# Autodesk Inventor assembly: Assembly1
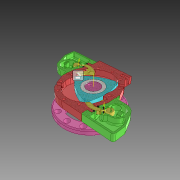
[picture p0: Inventor's stored thumbnail of the model, 180x180]
Saved by Autodesk Inventor 2020 (Build 240168000, 168)
## iProperties
Created: 2021-01-24
Part Number: Assembly1
Document SubType Name: Assembly
Designer: DDeGo
Author: DDeGo
## Documents named in this file (15)
- C:\Users\DDeGo\Documents\Drew\Projects\AirWankelEngine\cad\EngineAssembly.iam
- C:\Users\DDeGo\Documents\Drew\Projects\AirWankelEngine\cad\housing.ipt
- C:\Users\DDeGo\Documents\Drew\Projects\AirWankelEngine\cad\housingValve.ipt
- C:\Users\DDeGo\Documents\Drew\Projects\AirWankelEngine\cad\ValveFlapper.ipt
- C:\Users\DDeGo\Documents\Drew\Projects\AirWankelEngine\cad\housingPlate.ipt
- C:\Users\DDeGo\Documents\Drew\Projects\AirWankelEngine\cad\piston.ipt
- C:\Users\DDeGo\Documents\Drew\Projects\AirWankelEngine\cad\hardware\6701 bearing.ipt
- C:\Users\DDeGo\Documents\Drew\Projects\AirWankelEngine\cad\hardware\MR85 bearing.ipt
- C:\Users\DDeGo\Documents\Drew\Projects\AirWankelEngine\cad\camshaft.ipt
- C:\Users\DDeGo\Documents\Drew\Projects\AirWankelEngine\cad\CamPlate.ipt
- C:\Users\DDeGo\Documents\Drew\Projects\AirWankelEngine\cad\hardware\6mm bb.ipt
- C:\Users\DDeGo\Documents\Drew\Projects\AirWankelEngine\cad\hardware\oring_5x7.ipt
- C:\Users\DDeGo\Documents\Drew\Projects\AirWankelEngine\cad\Flywheel.ipt
- C:\Users\DDeGo\Documents\Drew\Projects\AirWankelEngine\cad\proto_clamp.ipt
- C:\Users\DDeGo\Documents\Drew\Projects\AirWankelEngine\cad\ValveSpring.ipt
## Components (22 placed, 14 different names)
1. housing:1 — Flush:1, Mate:1, Flush:2, Mate:2, Mate:3, Mate:9, Mate:10, Mate:14, Mate:15, Mate:18, Mate:22, Mate:25, Mate:26, Mate:27, Angle:1, Angle:2, Angle:3, Flush:4
2. housingValve:1 — Flush:1, Mate:1, Flush:2, Mate:28, Mate:31, Mate:35, Mate:36, Mate:37, Mate:38, Mate:39, Mate:43
3. ValveFlapper:1 — Mate:2, Mate:3, Flush:3, Valve2_flapper
4. piston:1 — Mate:7, Mate:8, Mate:14, Rotation:1, Angle:7
5. 6701 bearing:1 — Mate:7, Mate:8, Mate:13, Angle:7
6. MR85 bearing:1 — Mate:9, Mate:10, Mate:11, Mate:12
7. camshaft:1 — Mate:11, Mate:12, Mate:13, Mate:20, Mate:21, Rotation:1, Rotation:2, Piston
8. CamPlate:1 — Mate:20, Mate:21, Mate:32, Mate:33, Mate:34
9. housingPlate:2 — Mate:15, Mate:18, Mate:22, Mate:23, Mate:24
10. MR85 bearing:2 — Mate:23, Mate:24
11. 6mm bb:1 — Mate:28, Valve2_ball
12. housingValve:2 — Mate:26, Mate:27, Angle:1, Mate:29, Mate:40, Mate:41, Mate:42, Mate:44, Mate:45
13. ValveFlapper:2 — Mate:25, Flush:3, Valve1_flapper
14. 6mm bb:2 — Mate:29, Valve1_ball
15. oring_5x7:1 — Mate:44, Mate:45, Valve1_ball
16. oring_5x7:2 — Mate:31, Mate:43, Valve2_ball
17. oring_5x7:3 — Angle:2
18. oring_5x7:4 — Angle:3
19. Flywheel:1 — Mate:32, Mate:33, Mate:34, Rotation:2
20. proto_clamp:1 — Mate:35, Mate:36, Flush:4
21. ValveSpring:1 — Mate:37, Mate:38, Mate:39
22. ValveSpring:2 — Mate:40, Mate:41, Mate:42
## Relationships (53: Mate 40, Angle 7, Flush 4, RelateRotation 2)
- Flush:1: housing:1 ↔ housingValve:1
- Mate:1: housing:1 ↔ housingValve:1
- Flush:2: housing:1 ↔ housingValve:1
- Mate:2: housing:1 ↔ ValveFlapper:1
- Mate:3 (0.5 mm): housing:1 ↔ ValveFlapper:1
- Mate:7: piston:1 ↔ 6701 bearing:1
- Mate:8: piston:1 ↔ 6701 bearing:1
- Mate:9: housing:1 ↔ MR85 bearing:1
- Mate:10: housing:1 ↔ MR85 bearing:1
- Mate:11: MR85 bearing:1 ↔ camshaft:1
- Mate:12: MR85 bearing:1 ↔ camshaft:1
- Mate:13: 6701 bearing:1 ↔ camshaft:1
- Mate:14: housing:1 ↔ piston:1
- Mate:15: housing:1 ↔ housingPlate:2
- Mate:18: housing:1 ↔ housingPlate:2
- Mate:20: camshaft:1 ↔ CamPlate:1
- Mate:21: camshaft:1 ↔ CamPlate:1
- Mate:22: housing:1 ↔ housingPlate:2
- Mate:23: housingPlate:2 ↔ MR85 bearing:2
- Mate:24: housingPlate:2 ↔ MR85 bearing:2
- Mate:25: housing:1 ↔ ValveFlapper:2
- Flush:3: ValveFlapper:1 ↔ ValveFlapper:2
- Mate:26: housing:1 ↔ housingValve:2
- Mate:27: housing:1 ↔ housingValve:2
- Angle:1 (0 deg): housing:1 ↔ housingValve:2
- Mate:28: housingValve:1 ↔ 6mm bb:1
- Mate:29: housingValve:2 ↔ 6mm bb:2
- Mate:31: housingValve:1 ↔ oring_5x7:2
- Angle:2 (0 deg): housing:1 ↔ oring_5x7:3
- Angle:3 (0 deg): housing:1 ↔ oring_5x7:4
- Mate:32: CamPlate:1 ↔ Flywheel:1
- Mate:33: CamPlate:1 ↔ Flywheel:1
- Mate:34: CamPlate:1 ↔ Flywheel:1
- Mate:35: housingValve:1 ↔ proto_clamp:1
- Mate:36: housingValve:1 ↔ proto_clamp:1
- Flush:4: housing:1 ↔ proto_clamp:1
- Mate:37 (0.1 mm): housingValve:1 ↔ ValveSpring:1
- Mate:38 (0.1 mm): housingValve:1 ↔ ValveSpring:1
- Mate:39 (1 mm): housingValve:1 ↔ ValveSpring:1
- Mate:40 (0.1 mm): housingValve:2 ↔ ValveSpring:2
- Mate:41 (0.1 mm): housingValve:2 ↔ ValveSpring:2
- Mate:42 (1 mm): housingValve:2 ↔ ValveSpring:2
- Rotation:1 [RelateRotation] (3 ul): piston:1 ↔ camshaft:1
- Rotation:2 [RelateRotation] (1 ul): camshaft:1 ↔ Flywheel:1
- Mate:43: housingValve:1 ↔ oring_5x7:2
- Mate:44: housingValve:2 ↔ oring_5x7:1
- Mate:45: housingValve:2 ↔ oring_5x7:1
- Piston [Angle] (0 deg): camshaft:1
- Valve1_ball [Mate] (1.5 mm): 6mm bb:2 ↔ oring_5x7:1
- Valve1_flapper [Angle] (180 deg): ValveFlapper:2
- Valve2_ball [Mate] (1.5 mm): 6mm bb:1 ↔ oring_5x7:2
- Valve2_flapper [Angle] (-31 deg): ValveFlapper:1
- Angle:7 (0 deg): piston:1 ↔ 6701 bearing:1
